# Autodesk Inventor assembly: Robot
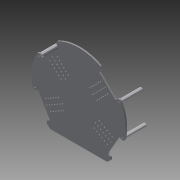
[picture p0: Inventor's stored thumbnail of the model, 180x180]
Saved by Autodesk Inventor 2015 (Build 190159000, 159)
## iProperties
Created: 2016-08-02
Part Number: Robot
Document SubType Name: Assembly
Designer: James Yelland
Author: James Yelland
## Documents named in this file (3)
- C:\Users\James Yelland\git\Layers-2017\Models\Robot.iam
- C:\Users\James Yelland\git\Layers-2017\Models\Bottom Plate.ipt
- C:\Users\James Yelland\git\Layers-2017\Models\Standoff 45.ipt
## Components (5 placed, 2 different names)
1. Bottom Plate:1 — Mate:1, Mate:2, Mate:3, Mate:4, Mate:5, Mate:6, Mate:7, Mate:8
2. Standoff 45:1 — Mate:2, Mate:7
3. Standoff 45:2 — Mate:1, Mate:5
4. Standoff 45:3 — Mate:3, Mate:6
5. Standoff 45:4 — Mate:4, Mate:8
## Relationships (8: Mate 8)
- Mate:1: Bottom Plate:1 ↔ Standoff 45:2
- Mate:2: Bottom Plate:1 ↔ Standoff 45:1
- Mate:3: Bottom Plate:1 ↔ Standoff 45:3
- Mate:4: Bottom Plate:1 ↔ Standoff 45:4
- Mate:5: Bottom Plate:1 ↔ Standoff 45:2
- Mate:6: Bottom Plate:1 ↔ Standoff 45:3
- Mate:7: Bottom Plate:1 ↔ Standoff 45:1
- Mate:8: Bottom Plate:1 ↔ Standoff 45:4
